# Autodesk Inventor assembly: Intake 3 Arm
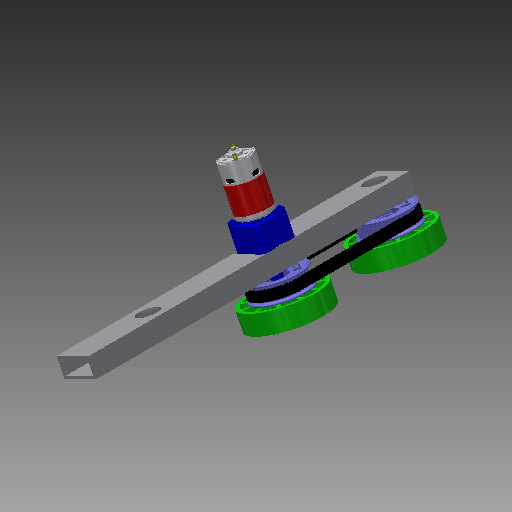
[picture p0: Inventor's stored thumbnail of the model, 512x512]
Saved by Autodesk Inventor 2018 (Build 220112000, 112)
## iProperties
Created: 2018-01-20
Part Number: Intake 3 Arm
Document SubType Name: Assembly
Designer: Apple
Author: Apple
## Documents named in this file (6)
- C:\Users\Apple\Documents\Inventor\2018 PowerUp\Cube Intake\Intake 3 Arm.iam
- C:\Users\Apple\Documents\Inventor\2018 PowerUp\Cube Intake\Sport57 with Redline and 4inc wheel.iam
- C:\Users\Apple\Documents\Inventor\2018 PowerUp\2018 Scissor\1x2 arm.ipt
- C:\Users\Apple\Documents\Inventor\2018 PowerUp\AndyMark\am-3480+4IN+500Hex+Bore+Compliant+Wheel.ipt
- C:\Users\Apple\Documents\Inventor\2018 PowerUp\AndyMark\42toothHTDpulleyHalfRev2.ipt
- C:\Users\Apple\Documents\Inventor\2018 PowerUp\Cube Intake\Belt.ipt
## Components (6 placed, 5 different names)
1. Sport57 with Redline and 4inc wheel:1 [sub-assembly] — Mate:1, Mate:2, Flush:2, Mate:12, Flush:3
2. 1x2 arm:1 — Mate:1, Mate:2, Mate:4, Mate:12
3. am-3480+4IN+500Hex+Bore+Compliant+Wheel:1 — Mate:4, Mate:8, Flush:2, Mate:11
4. 42toothHTDpulleyHalfRev2:1 — Mate:5, Mate:6, Mate:7, Mate:11
5. 42toothHTDpulleyHalfRev2:2 — Mate:5, Mate:6, Mate:7, Mate:8
6. Belt:1 — Flush:3
## Relationships (11: Mate 9, Flush 2)
- Mate:1: Sport57 with Redline and 4inc wheel:1 ↔ 1x2 arm:1
- Mate:2: Sport57 with Redline and 4inc wheel:1 ↔ 1x2 arm:1
- Mate:4: 1x2 arm:1 ↔ am-3480+4IN+500Hex+Bore+Compliant+Wheel:1
- Mate:5: 42toothHTDpulleyHalfRev2:1 ↔ 42toothHTDpulleyHalfRev2:2
- Mate:6: 42toothHTDpulleyHalfRev2:1 ↔ 42toothHTDpulleyHalfRev2:2
- Mate:7: 42toothHTDpulleyHalfRev2:1 ↔ 42toothHTDpulleyHalfRev2:2
- Mate:8: am-3480+4IN+500Hex+Bore+Compliant+Wheel:1 ↔ 42toothHTDpulleyHalfRev2:2
- Flush:2: Sport57 with Redline and 4inc wheel:1 ↔ am-3480+4IN+500Hex+Bore+Compliant+Wheel:1
- Mate:11: am-3480+4IN+500Hex+Bore+Compliant+Wheel:1 ↔ 42toothHTDpulleyHalfRev2:1
- Mate:12: Sport57 with Redline and 4inc wheel:1 ↔ 1x2 arm:1
- Flush:3: Sport57 with Redline and 4inc wheel:1 ↔ Belt:1
